# Autodesk Inventor assembly: bin
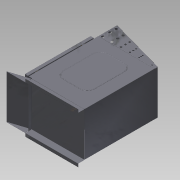
[picture p0: Inventor's stored thumbnail of the model, 180x180]
Saved by Autodesk Inventor 2012 (Build 160160000, 160)
## iProperties
Created: 2012-04-17
Part Number: bin
Document SubType Name: Assembly
Designer: thanos
Author: thanos
## Documents named in this file (10)
- C:\WORKSHOP\ADMETAL\sheet.metal.bin\predesign\bin.iam
- C:\WORKSHOP\ADMETAL\sheet.metal.bin\predesign\cap.ipt
- C:\WORKSHOP\ADMETAL\sheet.metal.bin\predesign\body.ipt
- C:\WORKSHOP\ADMETAL\sheet.metal.bin\predesign\Hinge\Hinge.iam
- C:\WORKSHOP\ADMETAL\sheet.metal.bin\predesign\door.ipt
- C:\WORKSHOP\ADMETAL\sheet.metal.bin\predesign\deck.ipt
- C:\WORKSHOP\ADMETAL\sheet.metal.bin\predesign\deck.incline.ipt
- C:\WORKSHOP\ADMETAL\sheet.metal.bin\predesign\bin.ipt
- C:\WORKSHOP\ADMETAL\sheet.metal.bin\predesign\wheel.ipt
- C:\WORKSHOP\ADMETAL\sheet.metal.bin\predesign\handle.ipt
## Components (13 placed, 9 different names)
1. cap:1 — Mate:1, Flush:1, Flush:2
2. body:1 — Mate:1, Flush:1, Flush:2, Mate:2, Flush:3, Flush:4, Mate:4, Mate:5, Flush:7, Flush:8, Mate:8
3. door:1 — Mate:3, Flush:4, Flush:6
4. Hinge:1 [sub-assembly] — Mate:2, Flush:3, Mate:3, Flush:5, Flush:6
5. Hinge:2 [sub-assembly] — Mate:4, Flush:5
6. deck:1 — Mate:5, Flush:7, Flush:8, Mate:6, Tangent:1, Tangent:2
7. deck.incline:1 — Mate:6
8. bin:1 — Mate:8, Flush:9, Flush:10, Mate:9, Mate:10, Flush:11
9. handle:1 — Mate:10, Flush:11
10. wheel:1 — Flush:9, Flush:10, Mate:9, Tangent:1
11. wheel:2 — Tangent:2
12. wheel:3
13. wheel:4
## Component patterns: (4 elements, first: wheel:1)
## Relationships (22: Flush 11, Mate 9, Tangent 2)
- Mate:1: cap:1 ↔ body:1
- Flush:1: cap:1 ↔ body:1
- Flush:2: cap:1 ↔ body:1
- Mate:2: body:1 ↔ Hinge:1
- Flush:3 (30 mm): body:1 ↔ Hinge:1
- Mate:3: door:1 ↔ Hinge:1
- Flush:4: body:1 ↔ door:1
- Mate:4: body:1 ↔ Hinge:2
- Flush:5: Hinge:1 ↔ Hinge:2
- Flush:6 (30 mm): door:1 ↔ Hinge:1
- Mate:5: body:1 ↔ deck:1
- Flush:7: body:1 ↔ deck:1
- Flush:8: body:1 ↔ deck:1
- Mate:6: deck:1 ↔ deck.incline:1
- Mate:8 (120 mm): body:1 ↔ bin:1
- Flush:9 (50 mm): bin:1 ↔ wheel:1
- Flush:10 (50 mm): bin:1 ↔ wheel:1
- Mate:9: bin:1 ↔ wheel:1
- Mate:10: bin:1 ↔ handle:1
- Flush:11 (200 mm): bin:1 ↔ handle:1
- Tangent:1: deck:1 ↔ wheel:1
- Tangent:2: deck:1 ↔ wheel:2
